# Autodesk Inventor assembly: BoreDevice_3
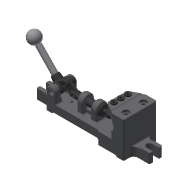
[picture p0: Inventor's stored thumbnail of the model, 180x180]
Saved by Autodesk Inventor 2022 Beta2 (Build 260130000, 130) ContinuousBuild 0
## iProperties
Created: 2006-01-30
Part Number: BoreDevice_3
Document SubType Name: Assembly
Designer: landrews
Author: landrews
## Documents named in this file (11)
- C:\Autodesk Inventor 2021 Intro Practice Files\BoreDevice_3.iam
- C:\Autodesk Inventor 2021 Intro Practice Files\Bore Base.ipt
- C:\Autodesk Inventor 2021 Intro Practice Files\Pin Pressure.ipt
- C:\Autodesk Inventor 2021 Intro Practice Files\Lever Angle.ipt
- C:\Autodesk Inventor 2021 Intro Practice Files\Fixutre Drill.ipt
- C:\Autodesk Inventor 2021 Intro Practice Files\Link_N.ipt
- C:\Autodesk Inventor 2021 Intro Practice Files\Thumb Screw.ipt
- C:\Autodesk Inventor 2021 Intro Practice Files\Screw Adjust.ipt
- C:\Autodesk Inventor 2021 Intro Practice Files\Pin Seized.ipt
- C:\Autodesk Inventor 2021 Intro Practice Files\Ball Lever.ipt
- C:\Autodesk Inventor 2021 Intro Practice Files\Bushing Drill.ipt
## Components (12 placed, 10 different names)
1. Bore Base:1 — Mate:2, Mate:3, Insert:5, Insert:6, Mate:5
2. Pin Pressure:1 — Mate:5, Mate:6, Mate:7, Mate:8
3. Lever Angle:1 — Mate:2, Mate:3, Insert:10, Mate:11, Mate:12
4. Link_N:1 — Insert:10, Mate:6
5. Screw Adjust:1 — Mate:9
6. Thumb Screw:1 — Mate:7, Mate:8, Mate:9
7. Pin Seized:1 — Mate:11, Mate:12, Insert:11
8. Ball Lever:1 — Insert:11
9. Fixutre Drill:1 — Insert:5, Insert:6, Insert:12, Insert:13, Insert:14
10. Bushing Drill:1 — Insert:12
11. Bushing Drill:2 — Insert:14
12. Bushing Drill:3 — Insert:13
## Relationships (16: Mate 9, Insert 7)
- Mate:2: Bore Base:1 ↔ Lever Angle:1
- Mate:3: Bore Base:1 ↔ Lever Angle:1
- Insert:5: Bore Base:1 ↔ Fixutre Drill:1
- Insert:6: Bore Base:1 ↔ Fixutre Drill:1
- Mate:5: Bore Base:1 ↔ Pin Pressure:1
- Insert:10: Lever Angle:1 ↔ Link_N:1
- Mate:6: Pin Pressure:1 ↔ Link_N:1
- Mate:7: Pin Pressure:1 ↔ Thumb Screw:1
- Mate:8: Pin Pressure:1 ↔ Thumb Screw:1
- Mate:9: Screw Adjust:1 ↔ Thumb Screw:1
- Mate:11: Lever Angle:1 ↔ Pin Seized:1
- Mate:12: Lever Angle:1 ↔ Pin Seized:1
- Insert:11: Pin Seized:1 ↔ Ball Lever:1
- Insert:12: Fixutre Drill:1 ↔ Bushing Drill:1
- Insert:13: Fixutre Drill:1 ↔ Bushing Drill:3
- Insert:14: Fixutre Drill:1 ↔ Bushing Drill:2
